# Autodesk Inventor assembly: CyberOrto
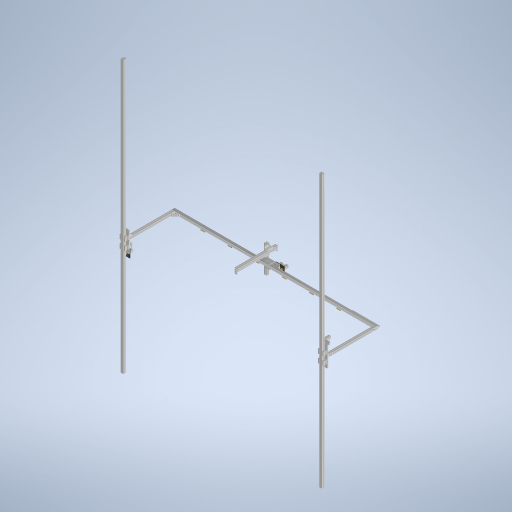
[picture p0: Inventor's stored thumbnail of the model, 512x512]
Saved by Autodesk Inventor 2023 (Build 270158000, 158)
## iProperties
RuleStatus: InUse
Created: 2021-12-29
Part Number: CyberOrto
Document SubType Name: Assembly
Designer: matte
Author: matte
## Documents named in this file (30)
- C:\Users\matte\Documents\GitHub\MDM-CyberOrto-CAD\CyberOrto.iam
- C:\Users\matte\Documents\GitHub\MDM-CyberOrto-CAD\Pezzi singoli\Supporto SX.ipt
- C:\Users\matte\Documents\GitHub\MDM-CyberOrto-CAD\Parker components\03-Brackets_Gussets_Plates\09-Machined Gussets\20-102.ipt
- C:\Users\matte\Documents\GitHub\MDM-CyberOrto-CAD\Parker components\02-Fasteners\10-Standard T-Nuts\20-050.ipt
- C:\Users\matte\Documents\GitHub\MDM-CyberOrto-CAD\Parker components\02-Fasteners\16-Screws\01-Metric Screws\01-Button Head\24-118-8.ipt
- C:\Users\matte\Documents\GitHub\MDM-CyberOrto-CAD\Guida a terra.iam
- C:\Users\matte\Documents\GitHub\MDM-CyberOrto-CAD\Parker components\05-Handles_Hinges\13-Pivot Joints\23-010.iam
- C:\Users\matte\Documents\GitHub\MDM-CyberOrto-CAD\Parker components\02-Fasteners\10-Standard T-Nuts\20-058.ipt
- C:\Users\matte\Documents\GitHub\MDM-CyberOrto-CAD\Parker components\02-Fasteners\16-Screws\01-Metric Screws\01-Button Head\24-116-8.ipt
- C:\Users\matte\Documents\GitHub\MDM-CyberOrto-CAD\Pezzi singoli\Supporto DX.ipt
- C:\Users\matte\Documents\GitHub\MDM-CyberOrto-CAD\Parker components\02-Fasteners\16-Screws\01-Metric Screws\01-Button Head\24-120-8.ipt
- C:\Users\matte\Documents\GitHub\MDM-CyberOrto-CAD\Pezzi singoli\Supporto lineare\Carrello semplice.iam
- C:\Users\matte\Documents\GitHub\MDM-CyberOrto-CAD\Platform.ipt
- C:\Users\matte\Documents\GitHub\MDM-CyberOrto-CAD\Parker components\02-Fasteners\16-Screws\01-Metric Screws\01-Button Head\24-130-6.ipt
- C:\Users\matte\Documents\GitHub\MDM-CyberOrto-CAD\Parker components\02-Fasteners\15-T-Bolts_Nuts_Washers\03-Washers\24-700-6.ipt
- C:\Users\matte\Documents\GitHub\MDM-CyberOrto-CAD\Parker components\02-Fasteners\15-T-Bolts_Nuts_Washers\02-Nuts\24-706-6.ipt
- C:\Users\matte\Documents\GitHub\MDM-CyberOrto-CAD\Servo Motor 50W\bch2mba531ca5c.ipt
- C:\Users\matte\Documents\GitHub\MDM-CyberOrto-CAD\Rack_Pinion\Rack gear scaled1.ipt
- C:\Users\matte\Documents\GitHub\MDM-CyberOrto-CAD\Rack_Pinion\pinion_scaled1.ipt
- C:\Users\matte\Documents\GitHub\MDM-CyberOrto-CAD\Inventor Support\Content Center Files\it-IT\ISO 1580\ISO 1580 - M4 x 12_.ipt
- C:\Users\matte\Documents\GitHub\MDM-CyberOrto-CAD\Inventor Support\Content Center Files\it-IT\AS 1474(1)\AS 1474 - M4(1).ipt
- C:\Users\matte\Documents\GitHub\MDM-CyberOrto-CAD\Trave a terra\Trave a terra.iam
- C:\Users\matte\Documents\GitHub\MDM-CyberOrto-CAD\Racks.iam
- C:\Users\matte\Documents\GitHub\MDM-CyberOrto-CAD\Parker components\02-Fasteners\16-Screws\01-Metric Screws\03-Socket Head\24-320-8SS.ipt
- C:\Users\matte\Documents\GitHub\MDM-CyberOrto-CAD\Parker components\02-Fasteners\10-Standard T-Nuts\20-058SS.ipt
- C:\Users\matte\Documents\GitHub\MDM-CyberOrto-CAD\Torretta.iam
- C:\Users\matte\Documents\GitHub\MDM-CyberOrto-CAD\Pezzi singoli\13-106_f.ipt
- C:\Users\matte\Documents\GitHub\MDM-CyberOrto-CAD\Pezzi singoli\13-513.ipt
- C:\Users\matte\Documents\GitHub\MDM-CyberOrto-CAD\Pezzi singoli\10-040.ipt
- C:\Users\matte\Documents\GitHub\MDM-CyberOrto-CAD\Rack_Pinion\Rack_series.iam
## Components (70 placed, 29 different names)
1. 10-040:1 — Allineato:147, Coincidente:266, Allineato:148
2. Supporto SX:1 — Coincidente:6, Allineato:3, Coincidente:7, Coincidente:15, Coincidente:16, Coincidente:23, Coincidente:28, Coincidente:29, Coincidente:30, Allineato:147, Coincidente:266, Allineato:148
3. Supporto DX:1 — Coincidente:45, Allineato:7, Allineato:8, Coincidente:48, Allineato:9, Allineato:10
4. Torretta:1 [sub-assembly] — Coincidente:258, Allineato:145
5. pinion_scaled1:3 — Coincidente:258
6. 13-106_f:1 — Coincidente:264, Allineato:145
7. 13-106_f:2 — Coincidente:263
8. 13-513:1 — Coincidente:264
9. 13-513:2 — Coincidente:263
10. Rack_series:1 [sub-assembly] — Coincidente:272, Angolo:9, Allineato:150, Allineato:151
11. Rack_series:2 [sub-assembly] — Coincidente:273, Allineato:152, Allineato:153
12. 24-118-8:3 — Coincidente:19, Coincidente:20
13. 24-118-8:4 — Coincidente:21, Coincidente:22
14. 20-050:2 — Coincidente:11, Coincidente:12
15. 24-118-8:1 — Coincidente:13, Coincidente:14
16. 24-118-8:2 — Coincidente:17, Coincidente:18
17. 20-102:1 — Coincidente:6, Allineato:3, Coincidente:8, Coincidente:9, Coincidente:11, Coincidente:12, Coincidente:13, Coincidente:14, Coincidente:17, Coincidente:18, Coincidente:19, Coincidente:20, Coincidente:21, Coincidente:22
18. 20-050:1 — Coincidente:7, Coincidente:8, Coincidente:9
19. 24-118-8:5 — Coincidente:31, Coincidente:32, Coincidente:33
20. 24-118-8:6 — Coincidente:34, Coincidente:35
21. 24-118-8:7 — Coincidente:38, Coincidente:39
22. 24-118-8:8 — Coincidente:36, Coincidente:37
23. Guida a terra:1 [sub-assembly] — Coincidente:15, Coincidente:16, Coincidente:23, Coincidente:32, Coincidente:33, Coincidente:34, Coincidente:35, Coincidente:36, Coincidente:37, Coincidente:38, Coincidente:39, Coincidente:138, Coincidente:139, Allineato:61, Coincidente:141, Coincidente:143, Coincidente:145, Coincidente:162, Coincidente:210, Allineato:115
24. 20-050:3 — Coincidente:27, Allineato:4, Coincidente:28, Coincidente:30, Coincidente:31
25. 20-050:4 — Coincidente:27, Allineato:4, Coincidente:29
26. 23-010:1 [sub-assembly] — Coincidente:43, Coincidente:44, Coincidente:45, Allineato:7, Allineato:8, Coincidente:46, Coincidente:47
27. 20-058:1 — Coincidente:42
28. 24-116-8:1 — Coincidente:42, Coincidente:43, Coincidente:44
29. 24-120-8:1 — Coincidente:46, Coincidente:47
30. 24-120-8:2 — Coincidente:51, Coincidente:52
31. Carrello semplice:1 [sub-assembly] — Coincidente:48, Allineato:9, Allineato:10, Coincidente:51, Coincidente:52, Angolo:2, Angolo:3, Angolo:4, Allineato:59, Coincidente:130
32. 24-706-6:8 — Coincidente:142, Coincidente:143
33. 24-706-6:7 — Coincidente:140, Coincidente:141
34. 24-706-6:6 — Coincidente:144, Coincidente:145
35. 24-700-6:8
36. 24-130-6:8 — Coincidente:146
37. 24-700-6:7
38. 24-130-6:7 — Coincidente:144
39. 24-700-6:6
40. 24-706-6:5 — Coincidente:146, Coincidente:162
41. 24-700-6:5
42. Platform:3 — Coincidente:138, Coincidente:139, Allineato:61, Coincidente:158, Coincidente:159, Coincidente:160, Coincidente:164, Coincidente:166, Coincidente:167, Coincidente:168
43. 24-130-6:5 — Coincidente:142
44. 24-130-6:6 — Coincidente:140
45. bch2mba531ca5c:2 — Coincidente:158, Coincidente:161, Coincidente:211
46. ISO 1580 M4 x 12:5 — Coincidente:161
47. AS 1474 - Metrico M4:5 — Coincidente:167
48. ISO 1580 M4 x 12:6 — Coincidente:159, Coincidente:163
49. AS 1474 - Metrico M4:6 — Coincidente:168
50. AS 1474 - Metrico M4:7 — Coincidente:165, Coincidente:166
51. ISO 1580 M4 x 12:7 — Coincidente:165
52. AS 1474 - Metrico M4:8 — Coincidente:163, Coincidente:164
53. ISO 1580 M4 x 12:8 — Coincidente:160
54. Trave a terra:1 [sub-assembly] — Angolo:2, Angolo:3, Angolo:4, Allineato:59, Coincidente:130, Allineato:149, Coincidente:272, Angolo:9, Allineato:150, Allineato:151
55. pinion_scaled1:2 — Coincidente:211
56. Trave a terra:2 [sub-assembly] — Coincidente:210, Allineato:115, Allineato:149, Coincidente:273, Allineato:152, Allineato:153
57. Racks:19 [sub-assembly]
58. Racks:20 [sub-assembly]
59. Racks:21 [sub-assembly]
60. Racks:22 [sub-assembly]
61. Racks:23 [sub-assembly]
62. Racks:24 [sub-assembly]
63. Rack gear scaled1:6 — Allineato:134, Allineato:137, Coincidente:255, Allineato:138
64. 24-320-8SS:11 — Coincidente:251
65. 24-320-8SS:12
66. 20-050:5 — Coincidente:251, Allineato:134, Coincidente:254
67. Rack gear scaled1:7 — Allineato:137, Coincidente:255, Allineato:138
68. 24-320-8SS:14 — Coincidente:254
69. 24-320-8SS:13 — Coincidente:256
70. 20-058SS:6 — Coincidente:256
## Relationships (124: Mate 88, Flush 24, Insert 8, Angle 4)
- [Mate]: 10-040:1
- [Mate]: 10-040:1
- [Mate]: 10-040:1
- Coincidente:6 [Mate]: Supporto SX:1 ↔ 20-102:1
- Allineato:3 [Flush]: Supporto SX:1 ↔ 20-102:1
- Coincidente:7 [Mate]: Supporto SX:1 ↔ 20-050:1
- Coincidente:8 [Mate]: 20-102:1 ↔ 20-050:1
- Coincidente:9 [Mate]: 20-102:1 ↔ 20-050:1
- Coincidente:11 [Mate]: 20-050:2 ↔ 20-102:1
- Coincidente:12 [Mate]: 20-050:2 ↔ 20-102:1
- Coincidente:13 [Mate]: 24-118-8:1 ↔ 20-102:1
- Coincidente:14 [Mate]: 24-118-8:1 ↔ 20-102:1
- Coincidente:15 [Mate]: Supporto SX:1 ↔ Guida a terra:1
- Coincidente:16 [Mate]: Supporto SX:1 ↔ Guida a terra:1
- Coincidente:17 [Mate]: 24-118-8:2 ↔ 20-102:1
- Coincidente:18 [Mate]: 24-118-8:2 ↔ 20-102:1
- Coincidente:19 [Mate]: 24-118-8:3 ↔ 20-102:1
- Coincidente:20 [Mate]: 24-118-8:3 ↔ 20-102:1
- Coincidente:21 [Mate]: 24-118-8:4 ↔ 20-102:1
- Coincidente:22 [Mate]: 24-118-8:4 ↔ 20-102:1
- Coincidente:23 [Mate]: Supporto SX:1 ↔ Guida a terra:1
- Coincidente:27 [Mate]: 20-050:3 ↔ 20-050:4
- Allineato:4 [Flush]: 20-050:3 ↔ 20-050:4
- Coincidente:28 [Mate]: Supporto SX:1 ↔ 20-050:3
- Coincidente:29 [Mate]: Supporto SX:1 ↔ 20-050:4
- Coincidente:30 [Mate]: Supporto SX:1 ↔ 20-050:3
- Coincidente:31 [Mate]: 24-118-8:5 ↔ 20-050:3
- Coincidente:32 [Mate]: 24-118-8:5 ↔ Guida a terra:1
- Coincidente:33 [Mate]: 24-118-8:5 ↔ Guida a terra:1
- Coincidente:34 [Mate]: 24-118-8:6 ↔ Guida a terra:1
- Coincidente:35 [Mate]: 24-118-8:6 ↔ Guida a terra:1
- Coincidente:36 [Mate]: 24-118-8:8 ↔ Guida a terra:1
- Coincidente:37 [Mate]: 24-118-8:8 ↔ Guida a terra:1
- Coincidente:38 [Mate]: 24-118-8:7 ↔ Guida a terra:1
- Coincidente:39 [Mate]: 24-118-8:7 ↔ Guida a terra:1
- Coincidente:42 [Mate]: 20-058:1 ↔ 24-116-8:1
- Coincidente:43 [Mate]: 23-010:1 ↔ 24-116-8:1
- Coincidente:44 [Mate]: 23-010:1 ↔ 24-116-8:1
- Coincidente:45 [Mate]: Supporto DX:1 ↔ 23-010:1
- Allineato:7 [Flush]: Supporto DX:1 ↔ 23-010:1
- Allineato:8 [Flush]: Supporto DX:1 ↔ 23-010:1
- Coincidente:46 [Mate]: 23-010:1 ↔ 24-120-8:1
- Coincidente:47 [Mate]: 23-010:1 ↔ 24-120-8:1
- Coincidente:48 [Mate]: Supporto DX:1 ↔ Carrello semplice:1
- Allineato:9 [Flush]: Supporto DX:1 ↔ Carrello semplice:1
- Allineato:10 [Flush]: Supporto DX:1 ↔ Carrello semplice:1
- Coincidente:51 [Mate]: 24-120-8:2 ↔ Carrello semplice:1
- Coincidente:52 [Mate]: 24-120-8:2 ↔ Carrello semplice:1
- Angolo:2 [Angle] (0 deg): Carrello semplice:1 ↔ Trave a terra:1
- Angolo:3 [Angle] (0 deg): Carrello semplice:1 ↔ Trave a terra:1
- Angolo:4 [Angle] (0 deg): Carrello semplice:1 ↔ Trave a terra:1
- Allineato:59 [Flush] (19 mm): Carrello semplice:1 ↔ Trave a terra:1
- Coincidente:130 [Mate] (20 mm): Carrello semplice:1 ↔ Trave a terra:1
- [Insert]: 24-700-6:5 ↔ 24-130-6:5
- [Insert]: 24-700-6:6 ↔ 24-130-6:6
- [Insert]: 24-700-6:7 ↔ 24-130-6:7
- [Insert]: 24-700-6:8 ↔ 24-130-6:8
- [Insert]: 24-700-6:8 ↔ Platform:3
- [Insert]: 24-700-6:7 ↔ Platform:3
- [Insert]: 24-700-6:5 ↔ Platform:3
- [Insert]: 24-700-6:6 ↔ Platform:3
- Coincidente:138 [Mate]: Guida a terra:1 ↔ Platform:3
- Coincidente:139 [Mate]: Guida a terra:1 ↔ Platform:3
- Allineato:61 [Flush]: Guida a terra:1 ↔ Platform:3
- Coincidente:140 [Mate]: 24-706-6:7 ↔ 24-130-6:6
- Coincidente:141 [Mate]: Guida a terra:1 ↔ 24-706-6:7
- Coincidente:142 [Mate]: 24-706-6:8 ↔ 24-130-6:5
- Coincidente:143 [Mate]: Guida a terra:1 ↔ 24-706-6:8
- Coincidente:144 [Mate]: 24-706-6:6 ↔ 24-130-6:7
- Coincidente:145 [Mate]: Guida a terra:1 ↔ 24-706-6:6
- Coincidente:146 [Mate]: 24-130-6:8 ↔ 24-706-6:5
- [Mate]: bch2mba531ca5c:2 ↔ ISO 1580 M4 x 12:5
- [Mate]: ISO 1580 M4 x 12:5 ↔ AS 1474 - Metrico M4:5
- [Mate]: bch2mba531ca5c:2 ↔ ISO 1580 M4 x 12:8
- [Mate]: bch2mba531ca5c:2 ↔ ISO 1580 M4 x 12:8
- [Mate]: AS 1474 - Metrico M4:6 ↔ ISO 1580 M4 x 12:8
- [Mate]: bch2mba531ca5c:2 ↔ ISO 1580 M4 x 12:7
- [Mate]: bch2mba531ca5c:2 ↔ ISO 1580 M4 x 12:7
- [Mate]: bch2mba531ca5c:2 ↔ ISO 1580 M4 x 12:6
- [Mate]: bch2mba531ca5c:2 ↔ ISO 1580 M4 x 12:6
- Coincidente:158 [Mate]: Platform:3 ↔ bch2mba531ca5c:2
- Coincidente:159 [Mate]: Platform:3 ↔ ISO 1580 M4 x 12:6
- Coincidente:160 [Mate]: Platform:3 ↔ ISO 1580 M4 x 12:8
- Coincidente:161 [Mate]: bch2mba531ca5c:2 ↔ ISO 1580 M4 x 12:5
- Coincidente:162 [Mate]: Guida a terra:1 ↔ 24-706-6:5
- Coincidente:163 [Mate]: ISO 1580 M4 x 12:6 ↔ AS 1474 - Metrico M4:8
- Coincidente:164 [Mate]: Platform:3 ↔ AS 1474 - Metrico M4:8
- Coincidente:165 [Mate]: AS 1474 - Metrico M4:7 ↔ ISO 1580 M4 x 12:7
- Coincidente:166 [Mate]: Platform:3 ↔ AS 1474 - Metrico M4:7
- Coincidente:167 [Mate]: Platform:3 ↔ AS 1474 - Metrico M4:5
- Coincidente:168 [Mate]: Platform:3 ↔ AS 1474 - Metrico M4:6
- Coincidente:210 [Mate] (20 mm): Guida a terra:1 ↔ Trave a terra:2
- Allineato:115 [Flush] (19 mm): Guida a terra:1 ↔ Trave a terra:2
- Coincidente:211 [Mate]: bch2mba531ca5c:2 ↔ pinion_scaled1:2
- [Mate]: Rack gear scaled1:6 ↔ 24-320-8SS:11
- [Flush]: Rack gear scaled1:6 ↔ 24-320-8SS:11
- [Mate]: Rack gear scaled1:6 ↔ 24-320-8SS:12
- [Flush]: Rack gear scaled1:6 ↔ 24-320-8SS:12
- Coincidente:251 [Mate]: 24-320-8SS:11 ↔ 20-050:5
- Allineato:134 [Flush] (-23.224 mm): Rack gear scaled1:6 ↔ 20-050:5
- [Mate]: Rack gear scaled1:7 ↔ 24-320-8SS:13
- [Flush]: Rack gear scaled1:7 ↔ 24-320-8SS:13
- [Mate]: Rack gear scaled1:7 ↔ 24-320-8SS:14
- [Flush]: Rack gear scaled1:7 ↔ 24-320-8SS:14
- Coincidente:254 [Mate]: 20-050:5 ↔ 24-320-8SS:14
- Allineato:137 [Flush]: Rack gear scaled1:6 ↔ Rack gear scaled1:7
- Coincidente:255 [Mate]: Rack gear scaled1:6 ↔ Rack gear scaled1:7
- Allineato:138 [Flush]: Rack gear scaled1:6 ↔ Rack gear scaled1:7
- Coincidente:256 [Mate]: 24-320-8SS:13 ↔ 20-058SS:6
- Coincidente:258 [Mate]: Torretta:1 ↔ pinion_scaled1:3
- Coincidente:263 [Mate]: 13-106_f:2 ↔ 13-513:2
- Coincidente:264 [Mate]: 13-106_f:1 ↔ 13-513:1
- Allineato:145 [Flush] (19 mm): Torretta:1 ↔ 13-106_f:1
- Allineato:147 [Flush]: 10-040:1 ↔ Supporto SX:1
- Coincidente:266 [Mate]: 10-040:1 ↔ Supporto SX:1
- Allineato:148 [Flush]: 10-040:1 ↔ Supporto SX:1
- Allineato:149 [Flush]: Trave a terra:1 ↔ Trave a terra:2
- Coincidente:272 [Mate]: Rack_series:1 ↔ Trave a terra:1
- Angolo:9 [Angle] (0 deg): Rack_series:1 ↔ Trave a terra:1
- Allineato:150 [Flush]: Rack_series:1 ↔ Trave a terra:1
- Allineato:151 [Flush] (12.5 mm): Rack_series:1 ↔ Trave a terra:1
- Coincidente:273 [Mate]: Rack_series:2 ↔ Trave a terra:2
- Allineato:152 [Flush]: Rack_series:2 ↔ Trave a terra:2
- Allineato:153 [Flush] (12.5 mm): Rack_series:2 ↔ Trave a terra:2
## Named parameters: L_piatto_guide = 240 mm, L_tracce_terra = 3980 mm, L_traccia_superiore = 3000 mm, H_supporto = 700 mm, d311_d115 = 0 mm, d312_d116_d115 = 0 mm, d313_d117_d115 = 0 mm, d314_d118_d115 = 0 mm, d315_d119 = 0 mm, d316_d120 = 0 mm, d317_d121 = 0 mm, d318_d122 = 0 mm, d333_d234 = 0 mm, d334_d235 = 0 mm, d335_d237 = 0 mm, d336_d238 = 0 mm, d337_d239 = 0 mm, d338_d241 = 0 mm, d339_d242 = 0 mm, d341_d245 = 0 mm, d342_d246 = 0 mm, d530_d495_d398_d369 = 0 mm, d531_d496_d399_d370 = 0 mm, d532_d497_d400_d371 = 0 mm, d533_d498_d401_d372 = 0 mm, d538_d530_d495_d398_d369 = 0 mm, d539_d531_d496_d399_d370 = 0 mm, d540_d532_d497_d400_d371 = 0 mm, d541_d533_d498_d401_d372 = 0 mm
